(part 1 of 2)
# Autodesk Inventor assembly: 0008-10-02 X Axis
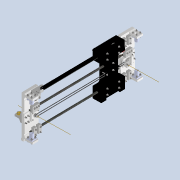
[picture p0: Inventor's stored thumbnail of the model, 180x180]
Saved by Autodesk Inventor 2020 (Build 240168000, 168)
## iProperties
Created: 2021-02-20
Part Number: 0008-10-02 X Axis
Document SubType Name: Assembly
Designer: Iulian Bors
Description: X axis
Author: Iulian Bors
Subject: 10-02
## Documents named in this file (36)
- Z:\I.A.B\Proiecte\0008 I.A.B 3D 2.1 Imprimanta aracet Metal\10 Mecanic\0008-10-02 X Axis.iam
- Z:\I.A.B\Proiecte\0008 I.A.B 3D 2.1 Imprimanta aracet Metal\10 Mecanic\0008-10-006 suport injectomat.ipt
- Z:\I.A.B\Proiecte\0008 I.A.B 3D 2.1 Imprimanta aracet Metal\10 Mecanic\0008-10-1009 LM10uu.ipt
- Z:\I.A.B\Proiecte\0008 I.A.B 3D 2.1 Imprimanta aracet Metal\10 Mecanic\0008-10-007 Contra suport injectomat.ipt
- Z:\I.A.B\Proiecte\0008 I.A.B 3D 2.1 Imprimanta aracet Metal\10 Mecanic\0008-10-008 X Axis suport.ipt
- Z:\I.A.B\Proiecte\0008 I.A.B 3D 2.1 Imprimanta aracet Metal\10 Mecanic\0008-10-1001 NEMA17 - Motor de passo.ipt
- Z:\I.A.B\Proiecte\0008 I.A.B 3D 2.1 Imprimanta aracet Metal\10 Mecanic\0008-10-1011 GT2 Timing Pulley 20 Tooth.ipt
- Z:\I.A.B\Proiecte\0008 I.A.B 3D 2.1 Imprimanta aracet Metal\10 Mecanic\0008-10-009 X Axis suport.ipt
- Z:\I.A.B\Proiecte\0008 I.A.B 3D 2.1 Imprimanta aracet Metal\10 Mecanic\0008-10-010 Fixare AxaX.ipt
- Z:\I.A.B\Proiecte\0008 I.A.B 3D 2.1 Imprimanta aracet Metal\10 Mecanic\0008-10-011 Fixare AxaX Mijloc.ipt
- Z:\I.A.B\Proiecte\0008 I.A.B 3D 2.1 Imprimanta aracet Metal\10 Mecanic\0008-10-012 Intinzator X.ipt
- Z:\I.A.B\Proiecte\0008 I.A.B 3D 2.1 Imprimanta aracet Metal\10 Mecanic\0008-10-1012 16T W6 B3 Without T_Shrinkwrap_1.ipt
- Z:\I.A.B\Proiecte\0008 I.A.B 3D 2.1 Imprimanta aracet Metal\10 Mecanic\0008-10-1013 LMK 10 Bearing.ipt
- Z:\I.A.B\Proiecte\0008 I.A.B 3D 2.1 Imprimanta aracet Metal\10 Mecanic\0008-10-013 Supăort Piulita Axa Z.ipt
- Z:\I.A.B\Proiecte\0008 I.A.B 3D 2.1 Imprimanta aracet Metal\10 Mecanic\0008-10-1004 Piulita.ipt
- Z:\I.A.B\Proiecte\0008 I.A.B 3D 2.1 Imprimanta aracet Metal\10 Mecanic\0008-10-1008 Bara 10_V1.ipt
- Z:\I.A.B\Proiecte\0008 I.A.B 3D 2.1 Imprimanta aracet Metal\20 Electric\0008-20-1003 Switch.ipt
- Z:\I.A.B\Proiecte\0008 I.A.B 3D 2.1 Imprimanta aracet Metal\10 Mecanic\0008-10-046 Fixare axa si port cablu.ipt
- Z:\I.A.B\Proiecte\0008 I.A.B 3D 2.1 Imprimanta aracet Metal\10 Mecanic\0008-10-2000 DIN 6912 - M4 x 25.ipt
- Z:\I.A.B\Proiecte\0008 I.A.B 3D 2.1 Imprimanta aracet Metal\10 Mecanic\0008-10-2002 DIN 125 - A 4.3.ipt
- Z:\I.A.B\Proiecte\0008 I.A.B 3D 2.1 Imprimanta aracet Metal\10 Mecanic\0008-10-2001 DIN 934 - M4 x 0.7.ipt
- Z:\I.A.B\Proiecte\0008 I.A.B 3D 2.1 Imprimanta aracet Metal\10 Mecanic\0008-10-2018 DIN 912 - M4 x 0.7 x 40.ipt
- Z:\I.A.B\Proiecte\0008 I.A.B 3D 2.1 Imprimanta aracet Metal\10 Mecanic\0008-10-2019 DIN 6912 - M4 x 50.ipt
- Z:\I.A.B\Proiecte\0008 I.A.B 3D 2.1 Imprimanta aracet Metal\10 Mecanic\0008-10-2003DIN 6912 - M4 x 35.ipt
- Z:\I.A.B\Proiecte\0008 I.A.B 3D 2.1 Imprimanta aracet Metal\10 Mecanic\0008-10-2006 DIN 7984 - M3 x 16.ipt
- Z:\I.A.B\Proiecte\0008 I.A.B 3D 2.1 Imprimanta aracet Metal\10 Mecanic\0008-10-2009 DIN 555-5 - M3.ipt
- Z:\I.A.B\Proiecte\0008 I.A.B 3D 2.1 Imprimanta aracet Metal\10 Mecanic\0008-10-2020 DIN 7991 - M3  x  16.ipt
- Z:\I.A.B\Proiecte\0008 I.A.B 3D 2.1 Imprimanta aracet Metal\10 Mecanic\0008-10-2005 DIN 125 - A 3.2.ipt
- Z:\I.A.B\Proiecte\0008 I.A.B 3D 2.1 Imprimanta aracet Metal\10 Mecanic\0008-10-2004 DIN 7984 - M3 x 20.ipt
- Z:\I.A.B\Proiecte\0008 I.A.B 3D 2.1 Imprimanta aracet Metal\10 Mecanic\0008-10-2021 DIN 7984 - M5 x 30.ipt
- Z:\I.A.B\Proiecte\0008 I.A.B 3D 2.1 Imprimanta aracet Metal\10 Mecanic\0008-10-2012 DIN 125 - A 5.3.ipt
- Z:\I.A.B\Proiecte\0008 I.A.B 3D 2.1 Imprimanta aracet Metal\10 Mecanic\0008-10-2022 DIN 934 - M5 x 0.8.ipt
- Z:\I.A.B\Proiecte\0008 I.A.B 3D 2.1 Imprimanta aracet Metal\10 Mecanic\0008-10-1023 Compress Spring11.ipt
- Z:\I.A.B\Proiecte\0008 I.A.B 3D 2.1 Imprimanta aracet Metal\10 Mecanic\Synchronous Belts Transmission1.iam
- Z:\I.A.B\Proiecte\0008 I.A.B 3D 2.1 Imprimanta aracet Metal\10 Mecanic\0008-10-1025 Wire chain.ipt
- Z:\I.A.B\Proiecte\0008 I.A.B 3D 2.1 Imprimanta aracet Metal\10 Mecanic\0008-10-04 Z axis_Shrinkwrap.ipt
## Components (326 placed, 35 different names)
1. 0008-10-006 suport injectomat.ipt:1 — Flush:3, Flush:4, Mate:8, Mate:9, Flush:5, Flush:6, Angle:2, Mate:17, Mate:23, Insert:178, Insert:197, Insert:198, Insert:199, Insert:200, Insert:201, Insert:202, Insert:212, Insert:213, Insert:214
2. 0008-10-1009 LM10uu.ipt:2 — Flush:1, Mate:5, Mate:8
3. 0008-10-1009 LM10uu.ipt:3 — Mate:5, Flush:121
4. 0008-10-1009 LM10uu.ipt:4 — Flush:4, Mate:6, Mate:9
5. 0008-10-1009 LM10uu.ipt:5 — Flush:3, Mate:6
6. 0008-10-007 Contra suport injectomat.ipt:6 — Flush:5, Flush:6, Mate:23, Flush:121, Flush:122, Insert:234, Insert:238, Mate:199, Flush:130, Insert:312, Insert:313, Flush:1
7. 0008-10-1008 Bara 10_V1.ipt:7
8. 0008-10-1008 Bara 10_V1.ipt:8 — Mate:188, Mate:189, Mate:191, Mate:192
9. 0008-10-009 X Axis suport.ipt:9 — Angle:2, Flush:10, Mate:21, Mate:22, Angle:3, Flush:26, Flush:27, Angle:4, Angle:5, Mate:26, Mate:27, Flush:32, Flush:34, Mate:38, Flush:36, Flush:37, Mate:164, Angle:28, Flush:127, Mate:194, Insert:49, Insert:50, Insert:51, Insert:52, Insert:140, Insert:141, Insert:142, Insert:143, Insert:156, Insert:157, Insert:158, Insert:159, Insert:172, Insert:173, Insert:174, Insert:289, Insert:290, Insert:291, Insert:292
10. 0008-10-008 X Axis suport.ipt:10 — Flush:10, Mate:21, Mate:30, Mate:31, Mate:33, Mate:34, Mate:35, Insert:21, Mate:172, Angle:25, Angle:29, Flush:128, Angle:30, Insert:65, Insert:66, Insert:67, Insert:68, Mate:196, Insert:91, Insert:98, Insert:99, Insert:109, Insert:110, Insert:111, Insert:124, Insert:125, Insert:126, Insert:127, Insert:302, Insert:303, Mate:197
11. 0008-10-1001 NEMA17 - Motor de passo.ipt:11 — Insert:1, Mate:22, Mate:26, Mate:27
12. 0008-10-1009 LM10uu.ipt:12 — Mate:17, Flush:122
13. 0008-10-1008 Bara 10_V1.ipt:13
14. 0008-10-1011 GT2 Timing Pulley 20 Tooth.ipt:14 — Insert:1, Flush:29, Flush:30, Angle:5
15. 0008-10-012 Intinzator X.ipt:15 — Flush:29, Insert:2, Angle:30, Insert:293, Insert:294
16. 0008-10-1012 16T W6 B3 Without T_Shrinkwrap_1.ipt:16 — Insert:2, Flush:30
17. 0008-10-1013 LMK 10 Bearing.ipt:17 — Mate:29, Angle:6, Mate:164
18. 0008-10-1013 LMK 10 Bearing.ipt:18 — Mate:33, Mate:34, Mate:35, Mate:202
19. 0008-10-1013 LMK 10 Bearing.ipt:19 — Mate:30, Mate:31, Angle:25, Insert:81, Insert:82, Insert:83, Insert:84
20. 0008-10-1013 LMK 10 Bearing.ipt:20 — Flush:32, Mate:29, Flush:34, Angle:6, Mate:194, Insert:23, Mate:195, Insert:35, Insert:36
21. 0008-10-046 Fixare axa si port cablu.ipt:21 — Angle:3, Flush:26, Insert:283, Insert:284, Insert:308, Insert:309, Mate:200, Flush:131, Flush:132
22. 0008-10-013 Supăort Piulita Axa Z.ipt:22 — Mate:38, Flush:36, Mate:39, Mate:40, Flush:37, Flush:38, Insert:218, Insert:228, Insert:229, Insert:230
23. 0008-10-1004 Piulita.ipt:23 — Mate:39, Mate:40, Flush:38, Insert:256, Insert:260, Insert:261, Insert:262
24. 0008-10-013 Supăort Piulita Axa Z.ipt:24 — Insert:21, Mate:172, Mate:173, Mate:174, Insert:251, Insert:252, Insert:253, Insert:254
25. 0008-10-1004 Piulita.ipt:25 — Mate:173, Mate:174, Insert:267, Insert:268, Insert:269, Insert:270, Mate:201
26. 0008-20-1003 Switch.ipt:28 — Mate:199, Flush:130, Insert:310, Insert:311
27. 0008-10-010 Fixare AxaX.ipt:29 — Mate:188, Angle:28, Flush:127, Mate:190
28. 0008-10-010 Fixare AxaX.ipt:30 — Mate:189, Mate:190
29. 0008-10-2020 DIN 7991 - M3  x  16.ipt:318 — Insert:309
30. 0008-10-2009 DIN 555-5 - M3.ipt:319
31. 0008-10-2005 DIN 125 - A 3.2.ipt:320
32. 0008-10-2020 DIN 7991 - M3  x  16.ipt:321 — Insert:308
33. 0008-10-2009 DIN 555-5 - M3.ipt:322
34. 0008-10-2005 DIN 125 - A 3.2.ipt:323
35. Synchronous Belts Transmission1.iam:324 [sub-assembly]
36. 0008-10-1025 Wire chain.ipt:325 — Mate:200, Flush:131, Flush:132
37. 0008-10-04 Z axis_Shrinkwrap.ipt:326 — Mate:201, Mate:202
38. 0008-10-2022 DIN 934 - M5 x 0.8.ipt:35 — Insert:295
39. 0008-10-2018 DIN 912 - M4 x 0.7 x 40.ipt:36 — Mate:198
40. 0008-10-2002 DIN 125 - A 4.3.ipt:37
41. 0008-10-2001 DIN 934 - M4 x 0.7.ipt:38
42. 0008-10-2002 DIN 125 - A 4.3.ipt:39 — Insert:302
43. 0008-10-2018 DIN 912 - M4 x 0.7 x 40.ipt:40
44. 0008-10-2002 DIN 125 - A 4.3.ipt:41
45. 0008-10-2001 DIN 934 - M4 x 0.7.ipt:42
46. 0008-10-2002 DIN 125 - A 4.3.ipt:43 — Insert:303
47. 0008-10-2003DIN 6912 - M4 x 35.ipt:44
48. 0008-10-2002 DIN 125 - A 4.3.ipt:45 — Insert:230
49. 0008-10-2002 DIN 125 - A 4.3.ipt:46
50. 0008-10-2001 DIN 934 - M4 x 0.7.ipt:47
51. 0008-10-2003DIN 6912 - M4 x 35.ipt:48
52. 0008-10-2002 DIN 125 - A 4.3.ipt:49 — Insert:229
53. 0008-10-2002 DIN 125 - A 4.3.ipt:50
54. 0008-10-2001 DIN 934 - M4 x 0.7.ipt:51
55. 0008-10-2003DIN 6912 - M4 x 35.ipt:52
56. 0008-10-2002 DIN 125 - A 4.3.ipt:53 — Insert:228
57. 0008-10-2002 DIN 125 - A 4.3.ipt:54
58. 0008-10-2001 DIN 934 - M4 x 0.7.ipt:55
59. 0008-10-2003DIN 6912 - M4 x 35.ipt:56
60. 0008-10-2002 DIN 125 - A 4.3.ipt:57 — Insert:234
61. 0008-10-2002 DIN 125 - A 4.3.ipt:58
62. 0008-10-2001 DIN 934 - M4 x 0.7.ipt:59
63. 0008-10-2003DIN 6912 - M4 x 35.ipt:60
64. 0008-10-2002 DIN 125 - A 4.3.ipt:61 — Insert:238
65. 0008-10-2002 DIN 125 - A 4.3.ipt:62
66. 0008-10-2001 DIN 934 - M4 x 0.7.ipt:63
67. 0008-10-2003DIN 6912 - M4 x 35.ipt:64
68. 0008-10-2002 DIN 125 - A 4.3.ipt:65 — Insert:253
69. 0008-10-2002 DIN 125 - A 4.3.ipt:66
70. 0008-10-2001 DIN 934 - M4 x 0.7.ipt:67
71. 0008-10-2003DIN 6912 - M4 x 35.ipt:68
72. 0008-10-2002 DIN 125 - A 4.3.ipt:69 — Insert:254
73. 0008-10-2002 DIN 125 - A 4.3.ipt:70
74. 0008-10-2001 DIN 934 - M4 x 0.7.ipt:71
75. 0008-10-2003DIN 6912 - M4 x 35.ipt:72
76. 0008-10-2002 DIN 125 - A 4.3.ipt:73 — Insert:252
77. 0008-10-2002 DIN 125 - A 4.3.ipt:74
78. 0008-10-2001 DIN 934 - M4 x 0.7.ipt:75
79. 0008-10-2003DIN 6912 - M4 x 35.ipt:76
80. 0008-10-2002 DIN 125 - A 4.3.ipt:77 — Insert:251
81. 0008-10-2002 DIN 125 - A 4.3.ipt:78
82. 0008-10-2001 DIN 934 - M4 x 0.7.ipt:79
83. 0008-10-2006 DIN 7984 - M3 x 16.ipt:80 — Insert:256
84. 0008-10-2009 DIN 555-5 - M3.ipt:81
85. 0008-10-2006 DIN 7984 - M3 x 16.ipt:82 — Insert:261
86. 0008-10-2009 DIN 555-5 - M3.ipt:83
87. 0008-10-2006 DIN 7984 - M3 x 16.ipt:84 — Insert:260
88. 0008-10-2009 DIN 555-5 - M3.ipt:85
89. 0008-10-2006 DIN 7984 - M3 x 16.ipt:86 — Insert:262
90. 0008-10-2009 DIN 555-5 - M3.ipt:87
91. 0008-10-2006 DIN 7984 - M3 x 16.ipt:88 — Insert:268
92. 0008-10-2009 DIN 555-5 - M3.ipt:89
93. 0008-10-2006 DIN 7984 - M3 x 16.ipt:90 — Insert:269
94. 0008-10-2009 DIN 555-5 - M3.ipt:91
95. 0008-10-2006 DIN 7984 - M3 x 16.ipt:92 — Insert:270
96. 0008-10-2009 DIN 555-5 - M3.ipt:93
97. 0008-10-2006 DIN 7984 - M3 x 16.ipt:94 — Insert:267
98. 0008-10-2009 DIN 555-5 - M3.ipt:95
99. 0008-10-2006 DIN 7984 - M3 x 16.ipt:96 — Insert:310
100. 0008-10-2006 DIN 7984 - M3 x 16.ipt:97 — Insert:311
101. 0008-10-2020 DIN 7991 - M3  x  16.ipt:98 — Insert:274, Insert:312
102. 0008-10-2009 DIN 555-5 - M3.ipt:99 — Insert:274
103. 0008-10-2005 DIN 125 - A 3.2.ipt:100
104. 0008-10-2020 DIN 7991 - M3  x  16.ipt:101 — Insert:313
105. 0008-10-2009 DIN 555-5 - M3.ipt:102
106. 0008-10-2005 DIN 125 - A 3.2.ipt:103
107. 0008-10-2020 DIN 7991 - M3  x  16.ipt:104 — Insert:283
108. 0008-10-2009 DIN 555-5 - M3.ipt:105
109. 0008-10-2005 DIN 125 - A 3.2.ipt:106
110. 0008-10-2020 DIN 7991 - M3  x  16.ipt:107 — Insert:284
111. 0008-10-2009 DIN 555-5 - M3.ipt:108
112. 0008-10-2005 DIN 125 - A 3.2.ipt:109
113. 0008-10-2004 DIN 7984 - M3 x 20.ipt:110 — Insert:285
114. 0008-10-2005 DIN 125 - A 3.2.ipt:111 — Insert:285, Insert:292
115. 0008-10-2004 DIN 7984 - M3 x 20.ipt:112
116. 0008-10-2005 DIN 125 - A 3.2.ipt:113 — Insert:291
117. 0008-10-2004 DIN 7984 - M3 x 20.ipt:114
118. 0008-10-2005 DIN 125 - A 3.2.ipt:115 — Insert:290
119. 0008-10-2004 DIN 7984 - M3 x 20.ipt:116
120. 0008-10-2005 DIN 125 - A 3.2.ipt:117 — Insert:289
121. 0008-10-2021 DIN 7984 - M5 x 30.ipt:118 — Insert:293
122. 0008-10-2012 DIN 125 - A 5.3.ipt:119 — Insert:294, Insert:295
123. 0008-10-2000 DIN 6912 - M4 x 25.ipt:120 — Insert:22, Insert:25
124. 0008-10-2002 DIN 125 - A 4.3.ipt:121 — Insert:22, Insert:23
125. 0008-10-2002 DIN 125 - A 4.3.ipt:122 — Insert:24
126. 0008-10-2001 DIN 934 - M4 x 0.7.ipt:123 — Insert:24, Insert:25
127. 0008-10-2000 DIN 6912 - M4 x 25.ipt:124
128. 0008-10-2002 DIN 125 - A 4.3.ipt:125 — Mate:195
129. 0008-10-2002 DIN 125 - A 4.3.ipt:126
130. 0008-10-2001 DIN 934 - M4 x 0.7.ipt:127
131. 0008-10-2000 DIN 6912 - M4 x 25.ipt:128
132. 0008-10-2002 DIN 125 - A 4.3.ipt:129 — Insert:36
133. 0008-10-2002 DIN 125 - A 4.3.ipt:130
134. 0008-10-2001 DIN 934 - M4 x 0.7.ipt:131
135. 0008-10-2000 DIN 6912 - M4 x 25.ipt:132
136. 0008-10-2002 DIN 125 - A 4.3.ipt:133 — Insert:35
137. 0008-10-2002 DIN 125 - A 4.3.ipt:134
138. 0008-10-2001 DIN 934 - M4 x 0.7.ipt:135
139. 0008-10-2000 DIN 6912 - M4 x 25.ipt:136
140. 0008-10-2002 DIN 125 - A 4.3.ipt:137 — Insert:50
141. 0008-10-2002 DIN 125 - A 4.3.ipt:138
142. 0008-10-2001 DIN 934 - M4 x 0.7.ipt:139
143. 0008-10-2000 DIN 6912 - M4 x 25.ipt:140
144. 0008-10-2002 DIN 125 - A 4.3.ipt:141 — Insert:52
145. 0008-10-2002 DIN 125 - A 4.3.ipt:142
146. 0008-10-2001 DIN 934 - M4 x 0.7.ipt:143
147. 0008-10-2000 DIN 6912 - M4 x 25.ipt:144
148. 0008-10-2002 DIN 125 - A 4.3.ipt:145 — Insert:51
149. 0008-10-2002 DIN 125 - A 4.3.ipt:146
150. 0008-10-2001 DIN 934 - M4 x 0.7.ipt:147
151. 0008-10-2000 DIN 6912 - M4 x 25.ipt:148
152. 0008-10-2002 DIN 125 - A 4.3.ipt:149 — Insert:49
153. 0008-10-2002 DIN 125 - A 4.3.ipt:150
154. 0008-10-2001 DIN 934 - M4 x 0.7.ipt:151
155. 0008-10-2000 DIN 6912 - M4 x 25.ipt:152
156. 0008-10-2002 DIN 125 - A 4.3.ipt:153 — Insert:66
157. 0008-10-2002 DIN 125 - A 4.3.ipt:154
158. 0008-10-2001 DIN 934 - M4 x 0.7.ipt:155
159. 0008-10-2000 DIN 6912 - M4 x 25.ipt:156
160. 0008-10-2002 DIN 125 - A 4.3.ipt:157 — Insert:65
161. 0008-10-2002 DIN 125 - A 4.3.ipt:158
162. 0008-10-2001 DIN 934 - M4 x 0.7.ipt:159
163. 0008-10-2000 DIN 6912 - M4 x 25.ipt:160
164. 0008-10-2002 DIN 125 - A 4.3.ipt:161 — Insert:67
165. 0008-10-2002 DIN 125 - A 4.3.ipt:162
166. 0008-10-2001 DIN 934 - M4 x 0.7.ipt:163
167. 0008-10-2000 DIN 6912 - M4 x 25.ipt:164
168. 0008-10-2002 DIN 125 - A 4.3.ipt:165 — Insert:68
169. 0008-10-2002 DIN 125 - A 4.3.ipt:166
170. 0008-10-2001 DIN 934 - M4 x 0.7.ipt:167
171. 0008-10-2000 DIN 6912 - M4 x 25.ipt:168
172. 0008-10-2002 DIN 125 - A 4.3.ipt:169 — Insert:84
173. 0008-10-2002 DIN 125 - A 4.3.ipt:170
174. 0008-10-2001 DIN 934 - M4 x 0.7.ipt:171
175. 0008-10-2000 DIN 6912 - M4 x 25.ipt:172
176. 0008-10-2002 DIN 125 - A 4.3.ipt:173 — Insert:83
177. 0008-10-2002 DIN 125 - A 4.3.ipt:174
178. 0008-10-2001 DIN 934 - M4 x 0.7.ipt:175
179. 0008-10-2000 DIN 6912 - M4 x 25.ipt:176
180. 0008-10-2002 DIN 125 - A 4.3.ipt:177 — Insert:82
181. 0008-10-2002 DIN 125 - A 4.3.ipt:178
182. 0008-10-2001 DIN 934 - M4 x 0.7.ipt:179
183. 0008-10-2000 DIN 6912 - M4 x 25.ipt:180
184. 0008-10-2002 DIN 125 - A 4.3.ipt:181 — Insert:81
185. 0008-10-2002 DIN 125 - A 4.3.ipt:182
186. 0008-10-2001 DIN 934 - M4 x 0.7.ipt:183
187. 0008-10-2018 DIN 912 - M4 x 0.7 x 40.ipt:184 — Insert:86, Insert:87
188. 0008-10-2002 DIN 125 - A 4.3.ipt:185
189. 0008-10-2001 DIN 934 - M4 x 0.7.ipt:186 — Insert:87
190. 0008-10-2002 DIN 125 - A 4.3.ipt:187 — Insert:86, Mate:196
191. 0008-10-2018 DIN 912 - M4 x 0.7 x 40.ipt:188
192. 0008-10-2002 DIN 125 - A 4.3.ipt:189
193. 0008-10-2001 DIN 934 - M4 x 0.7.ipt:190
194. 0008-10-2002 DIN 125 - A 4.3.ipt:191 — Insert:91
195. 0008-10-2018 DIN 912 - M4 x 0.7 x 40.ipt:192
196. 0008-10-2002 DIN 125 - A 4.3.ipt:193
197. 0008-10-2001 DIN 934 - M4 x 0.7.ipt:194
198. 0008-10-2002 DIN 125 - A 4.3.ipt:195 — Insert:98
199. 0008-10-2018 DIN 912 - M4 x 0.7 x 40.ipt:196
200. 0008-10-2002 DIN 125 - A 4.3.ipt:197
201. 0008-10-2001 DIN 934 - M4 x 0.7.ipt:198
202. 0008-10-2002 DIN 125 - A 4.3.ipt:199 — Insert:99
203. 0008-10-2018 DIN 912 - M4 x 0.7 x 40.ipt:200
204. 0008-10-2002 DIN 125 - A 4.3.ipt:201
205. 0008-10-2001 DIN 934 - M4 x 0.7.ipt:202
206. 0008-10-2002 DIN 125 - A 4.3.ipt:203 — Insert:110
207. 0008-10-2018 DIN 912 - M4 x 0.7 x 40.ipt:204
208. 0008-10-2002 DIN 125 - A 4.3.ipt:205
209. 0008-10-2001 DIN 934 - M4 x 0.7.ipt:206
210. 0008-10-2002 DIN 125 - A 4.3.ipt:207 — Insert:111
211. 0008-10-2018 DIN 912 - M4 x 0.7 x 40.ipt:208
212. 0008-10-2002 DIN 125 - A 4.3.ipt:209
213. 0008-10-2001 DIN 934 - M4 x 0.7.ipt:210
214. 0008-10-2002 DIN 125 - A 4.3.ipt:211 — Insert:109
215. 0008-10-2018 DIN 912 - M4 x 0.7 x 40.ipt:212
216. 0008-10-2002 DIN 125 - A 4.3.ipt:213
217. 0008-10-2001 DIN 934 - M4 x 0.7.ipt:214
218. 0008-10-2002 DIN 125 - A 4.3.ipt:215 — Insert:126
219. 0008-10-2018 DIN 912 - M4 x 0.7 x 40.ipt:216
220. 0008-10-2002 DIN 125 - A 4.3.ipt:217
221. 0008-10-2001 DIN 934 - M4 x 0.7.ipt:218
222. 0008-10-2002 DIN 125 - A 4.3.ipt:219 — Insert:124
223. 0008-10-2018 DIN 912 - M4 x 0.7 x 40.ipt:220
224. 0008-10-2002 DIN 125 - A 4.3.ipt:221
225. 0008-10-2001 DIN 934 - M4 x 0.7.ipt:222
226. 0008-10-2002 DIN 125 - A 4.3.ipt:223 — Insert:125
227. 0008-10-2018 DIN 912 - M4 x 0.7 x 40.ipt:224
228. 0008-10-2002 DIN 125 - A 4.3.ipt:225
229. 0008-10-2001 DIN 934 - M4 x 0.7.ipt:226
230. 0008-10-2002 DIN 125 - A 4.3.ipt:227 — Insert:127
231. 0008-10-2018 DIN 912 - M4 x 0.7 x 40.ipt:228
232. 0008-10-2002 DIN 125 - A 4.3.ipt:229
233. 0008-10-2001 DIN 934 - M4 x 0.7.ipt:230
234. 0008-10-2002 DIN 125 - A 4.3.ipt:231 — Insert:141
235. 0008-10-2018 DIN 912 - M4 x 0.7 x 40.ipt:232
236. 0008-10-2002 DIN 125 - A 4.3.ipt:233
237. 0008-10-2001 DIN 934 - M4 x 0.7.ipt:234
238. 0008-10-2002 DIN 125 - A 4.3.ipt:235 — Insert:142
239. 0008-10-2018 DIN 912 - M4 x 0.7 x 40.ipt:236
240. 0008-10-2002 DIN 125 - A 4.3.ipt:237
241. 0008-10-2001 DIN 934 - M4 x 0.7.ipt:238
242. 0008-10-2002 DIN 125 - A 4.3.ipt:239 — Insert:143
243. 0008-10-2018 DIN 912 - M4 x 0.7 x 40.ipt:240
244. 0008-10-2002 DIN 125 - A 4.3.ipt:241
245. 0008-10-2001 DIN 934 - M4 x 0.7.ipt:242
246. 0008-10-2002 DIN 125 - A 4.3.ipt:243 — Insert:140
247. 0008-10-2018 DIN 912 - M4 x 0.7 x 40.ipt:244
248. 0008-10-2002 DIN 125 - A 4.3.ipt:245
249. 0008-10-2001 DIN 934 - M4 x 0.7.ipt:246
250. 0008-10-2002 DIN 125 - A 4.3.ipt:247 — Insert:156
251. 0008-10-2018 DIN 912 - M4 x 0.7 x 40.ipt:248
252. 0008-10-2002 DIN 125 - A 4.3.ipt:249
253. 0008-10-2001 DIN 934 - M4 x 0.7.ipt:250
254. 0008-10-2002 DIN 125 - A 4.3.ipt:251 — Insert:157
255. 0008-10-2018 DIN 912 - M4 x 0.7 x 40.ipt:252
256. 0008-10-2002 DIN 125 - A 4.3.ipt:253
257. 0008-10-2001 DIN 934 - M4 x 0.7.ipt:254
258. 0008-10-2002 DIN 125 - A 4.3.ipt:255 — Insert:158
259. 0008-10-2018 DIN 912 - M4 x 0.7 x 40.ipt:256
260. 0008-10-2002 DIN 125 - A 4.3.ipt:257
261. 0008-10-2001 DIN 934 - M4 x 0.7.ipt:258
262. 0008-10-2002 DIN 125 - A 4.3.ipt:259 — Insert:159
263. 0008-10-2018 DIN 912 - M4 x 0.7 x 40.ipt:260
264. 0008-10-2002 DIN 125 - A 4.3.ipt:261
265. 0008-10-2001 DIN 934 - M4 x 0.7.ipt:262
266. 0008-10-2002 DIN 125 - A 4.3.ipt:263 — Insert:173
267. 0008-10-2018 DIN 912 - M4 x 0.7 x 40.ipt:264
268. 0008-10-2002 DIN 125 - A 4.3.ipt:265
269. 0008-10-2001 DIN 934 - M4 x 0.7.ipt:266
270. 0008-10-2002 DIN 125 - A 4.3.ipt:267 — Insert:174
271. 0008-10-2018 DIN 912 - M4 x 0.7 x 40.ipt:268
272. 0008-10-2002 DIN 125 - A 4.3.ipt:269
273. 0008-10-2001 DIN 934 - M4 x 0.7.ipt:270
274. 0008-10-2002 DIN 125 - A 4.3.ipt:271 — Insert:172
275. 0008-10-2019 DIN 6912 - M4 x 50.ipt:272 — Insert:175, Insert:177
276. 0008-10-2002 DIN 125 - A 4.3.ipt:273 — Insert:175, Insert:178
277. 0008-10-2002 DIN 125 - A 4.3.ipt:274 — Insert:176
278. 0008-10-2001 DIN 934 - M4 x 0.7.ipt:275 — Insert:176, Insert:177
279. 0008-10-2019 DIN 6912 - M4 x 50.ipt:276
280. 0008-10-2002 DIN 125 - A 4.3.ipt:277 — Insert:197
281. 0008-10-2002 DIN 125 - A 4.3.ipt:278
282. 0008-10-2001 DIN 934 - M4 x 0.7.ipt:279
283. 0008-10-2019 DIN 6912 - M4 x 50.ipt:280
284. 0008-10-2002 DIN 125 - A 4.3.ipt:281 — Insert:199
285. 0008-10-2002 DIN 125 - A 4.3.ipt:282
286. 0008-10-2001 DIN 934 - M4 x 0.7.ipt:283
287. 0008-10-2019 DIN 6912 - M4 x 50.ipt:284
288. 0008-10-2002 DIN 125 - A 4.3.ipt:285 — Insert:198
289. 0008-10-2002 DIN 125 - A 4.3.ipt:286
290. 0008-10-2001 DIN 934 - M4 x 0.7.ipt:287
291. 0008-10-2019 DIN 6912 - M4 x 50.ipt:288
292. 0008-10-2002 DIN 125 - A 4.3.ipt:289 — Insert:200
293. 0008-10-2002 DIN 125 - A 4.3.ipt:290
294. 0008-10-2001 DIN 934 - M4 x 0.7.ipt:291
295. 0008-10-2019 DIN 6912 - M4 x 50.ipt:292
296. 0008-10-2002 DIN 125 - A 4.3.ipt:293 — Insert:201
297. 0008-10-2002 DIN 125 - A 4.3.ipt:294
298. 0008-10-2001 DIN 934 - M4 x 0.7.ipt:295
299. 0008-10-2019 DIN 6912 - M4 x 50.ipt:296
300. 0008-10-2002 DIN 125 - A 4.3.ipt:297 — Insert:202
301. 0008-10-2002 DIN 125 - A 4.3.ipt:298
302. 0008-10-2001 DIN 934 - M4 x 0.7.ipt:299
303. 0008-10-2019 DIN 6912 - M4 x 50.ipt:300
304. 0008-10-2002 DIN 125 - A 4.3.ipt:301 — Insert:213
305. 0008-10-2002 DIN 125 - A 4.3.ipt:302
306. 0008-10-2001 DIN 934 - M4 x 0.7.ipt:303
307. 0008-10-2019 DIN 6912 - M4 x 50.ipt:304
308. 0008-10-2002 DIN 125 - A 4.3.ipt:305 — Insert:212
309. 0008-10-2002 DIN 125 - A 4.3.ipt:306
310. 0008-10-2001 DIN 934 - M4 x 0.7.ipt:307
311. 0008-10-2019 DIN 6912 - M4 x 50.ipt:308
312. 0008-10-2002 DIN 125 - A 4.3.ipt:309 — Insert:214
313. 0008-10-2002 DIN 125 - A 4.3.ipt:310
314. 0008-10-2001 DIN 934 - M4 x 0.7.ipt:311
315. 0008-10-2003DIN 6912 - M4 x 35.ipt:312 — Insert:215, Insert:217
316. 0008-10-2002 DIN 125 - A 4.3.ipt:313 — Insert:215, Insert:218
317. 0008-10-2002 DIN 125 - A 4.3.ipt:314 — Insert:216
318. 0008-10-2001 DIN 934 - M4 x 0.7.ipt:315 — Insert:216, Insert:217
319. 0008-10-011 Fixare AxaX Mijloc.ipt:26 — Flush:27, Angle:4
320. 0008-10-011 Fixare AxaX Mijloc.ipt:27
321. 0008-10-010 Fixare AxaX.ipt:31 — Mate:191, Angle:29, Flush:128, Flush:129, Mate:193
322. 0008-10-010 Fixare AxaX.ipt:32 — Mate:192, Flush:129, Mate:193
323. 0008-10-010 Fixare AxaX.ipt:33
324. 0008-10-010 Fixare AxaX.ipt:34
325. 0008-10-1023 Compress Spring11.ipt:316 — Mate:197, Mate:198
326. 0008-10-1023 Compress Spring11.ipt:317
## Component patterns: (2 elements, first: 0008-10-011 Fixare AxaX Mijloc.ipt:26), (2 elements, first: 0008-10-010 Fixare AxaX.ipt:31 + 0008-10-010 Fixare AxaX.ipt:32), (2 elements, first: 0008-10-1023 Compress Spring11.ipt:316)
## Relationships (368: Insert 288, Mate 43, Flush 27, Angle 9, Tangent 1)
- Flush:1 (20 mm): 0008-10-1009 LM10uu.ipt:2 ↔ 0008-10-007 Contra suport injectomat.ipt:6
- Mate:5: 0008-10-1009 LM10uu.ipt:2 ↔ 0008-10-1009 LM10uu.ipt:3
- Flush:3 (20 mm): 0008-10-006 suport injectomat.ipt:1 ↔ 0008-10-1009 LM10uu.ipt:5
- Flush:4 (20 mm): 0008-10-006 suport injectomat.ipt:1 ↔ 0008-10-1009 LM10uu.ipt:4
- Mate:6: 0008-10-1009 LM10uu.ipt:4 ↔ 0008-10-1009 LM10uu.ipt:5
- Mate:8: 0008-10-006 suport injectomat.ipt:1 ↔ 0008-10-1009 LM10uu.ipt:2
- Mate:9: 0008-10-006 suport injectomat.ipt:1 ↔ 0008-10-1009 LM10uu.ipt:4
- Flush:5: 0008-10-006 suport injectomat.ipt:1 ↔ 0008-10-007 Contra suport injectomat.ipt:6
- Flush:6: 0008-10-006 suport injectomat.ipt:1 ↔ 0008-10-007 Contra suport injectomat.ipt:6
- [Mate]: 0008-10-1009 LM10uu.ipt:3 ↔ 0008-10-1008 Bara 10_V1.ipt:7
- [Mate]: 0008-10-1009 LM10uu.ipt:5 ↔ 0008-10-1008 Bara 10_V1.ipt:8
- [Flush]: 0008-10-1008 Bara 10_V1.ipt:7 ↔ 0008-10-1008 Bara 10_V1.ipt:8
- [Tangent] (-3 mm): 0008-10-1008 Bara 10_V1.ipt:7 ↔ 0008-10-009 X Axis suport.ipt:9
- Angle:2 (0 deg): 0008-10-006 suport injectomat.ipt:1 ↔ 0008-10-009 X Axis suport.ipt:9
- [Flush] (-30 mm): 0008-10-1008 Bara 10_V1.ipt:7 ↔ 0008-10-009 X Axis suport.ipt:9
- Flush:10: 0008-10-009 X Axis suport.ipt:9 ↔ 0008-10-008 X Axis suport.ipt:10
- [Flush] (-30 mm): 0008-10-1008 Bara 10_V1.ipt:7 ↔ 0008-10-008 X Axis suport.ipt:10
- Mate:21: 0008-10-009 X Axis suport.ipt:9 ↔ 0008-10-008 X Axis suport.ipt:10
- Mate:17: 0008-10-006 suport injectomat.ipt:1 ↔ 0008-10-1009 LM10uu.ipt:12
- Insert:1: 0008-10-1001 NEMA17 - Motor de passo.ipt:11 ↔ 0008-10-1011 GT2 Timing Pulley 20 Tooth.ipt:14
- Mate:22 (-10 mm): 0008-10-009 X Axis suport.ipt:9 ↔ 0008-10-1001 NEMA17 - Motor de passo.ipt:11
- Mate:23 (2 mm): 0008-10-006 suport injectomat.ipt:1 ↔ 0008-10-007 Contra suport injectomat.ipt:6
- [Flush]: 0008-10-1008 Bara 10_V1.ipt:7 ↔ 0008-10-1008 Bara 10_V1.ipt:13
- [Mate]: 0008-10-1008 Bara 10_V1.ipt:7 ↔ 0008-10-046 Fixare axa si port cablu.ipt:21
- Angle:3 (0 deg): 0008-10-009 X Axis suport.ipt:9 ↔ 0008-10-046 Fixare axa si port cablu.ipt:21
- Flush:26 (35 mm): 0008-10-009 X Axis suport.ipt:9 ↔ 0008-10-046 Fixare axa si port cablu.ipt:21
- [Mate]: 0008-10-1008 Bara 10_V1.ipt:13 ↔ 0008-10-011 Fixare AxaX Mijloc.ipt:26
- Flush:27 (30 mm): 0008-10-009 X Axis suport.ipt:9 ↔ 0008-10-011 Fixare AxaX Mijloc.ipt:26
- Angle:4 (0 deg): 0008-10-009 X Axis suport.ipt:9 ↔ 0008-10-011 Fixare AxaX Mijloc.ipt:26
- Flush:29: 0008-10-1011 GT2 Timing Pulley 20 Tooth.ipt:14 ↔ 0008-10-012 Intinzator X.ipt:15
- Insert:2 (0.25 mm): 0008-10-012 Intinzator X.ipt:15 ↔ 0008-10-1012 16T W6 B3 Without T_Shrinkwrap_1.ipt:16
- Flush:30: 0008-10-1011 GT2 Timing Pulley 20 Tooth.ipt:14 ↔ 0008-10-1012 16T W6 B3 Without T_Shrinkwrap_1.ipt:16
- Angle:5 (0 deg): 0008-10-009 X Axis suport.ipt:9 ↔ 0008-10-1011 GT2 Timing Pulley 20 Tooth.ipt:14
- Mate:26 (1 mm): 0008-10-009 X Axis suport.ipt:9 ↔ 0008-10-1001 NEMA17 - Motor de passo.ipt:11
- Mate:27 (1 mm): 0008-10-009 X Axis suport.ipt:9 ↔ 0008-10-1001 NEMA17 - Motor de passo.ipt:11
- Flush:32 (15 mm): 0008-10-009 X Axis suport.ipt:9 ↔ 0008-10-1013 LMK 10 Bearing.ipt:20
- Mate:29: 0008-10-1013 LMK 10 Bearing.ipt:17 ↔ 0008-10-1013 LMK 10 Bearing.ipt:20
- Flush:34: 0008-10-009 X Axis suport.ipt:9 ↔ 0008-10-1013 LMK 10 Bearing.ipt:20
- Angle:6 (0 deg): 0008-10-1013 LMK 10 Bearing.ipt:17 ↔ 0008-10-1013 LMK 10 Bearing.ipt:20
- Mate:30: 0008-10-008 X Axis suport.ipt:10 ↔ 0008-10-1013 LMK 10 Bearing.ipt:19
- Mate:31: 0008-10-008 X Axis suport.ipt:10 ↔ 0008-10-1013 LMK 10 Bearing.ipt:19
- Mate:33: 0008-10-008 X Axis suport.ipt:10 ↔ 0008-10-1013 LMK 10 Bearing.ipt:18
- Mate:34: 0008-10-008 X Axis suport.ipt:10 ↔ 0008-10-1013 LMK 10 Bearing.ipt:18
- Mate:35: 0008-10-008 X Axis suport.ipt:10 ↔ 0008-10-1013 LMK 10 Bearing.ipt:18
- Mate:38: 0008-10-009 X Axis suport.ipt:9 ↔ 0008-10-013 Supăort Piulita Axa Z.ipt:22
- Flush:36: 0008-10-009 X Axis suport.ipt:9 ↔ 0008-10-013 Supăort Piulita Axa Z.ipt:22
- Mate:39: 0008-10-013 Supăort Piulita Axa Z.ipt:22 ↔ 0008-10-1004 Piulita.ipt:23
- Mate:40 (-12 mm): 0008-10-013 Supăort Piulita Axa Z.ipt:22 ↔ 0008-10-1004 Piulita.ipt:23
- Flush:37 (80 mm): 0008-10-009 X Axis suport.ipt:9 ↔ 0008-10-013 Supăort Piulita Axa Z.ipt:22
- Flush:38 (15 mm): 0008-10-013 Supăort Piulita Axa Z.ipt:22 ↔ 0008-10-1004 Piulita.ipt:23
- [Mate]: 0008-10-1008 Bara 10_V1.ipt:7 ↔ 0008-10-009 X Axis suport.ipt:9
- Mate:164: 0008-10-009 X Axis suport.ipt:9 ↔ 0008-10-1013 LMK 10 Bearing.ipt:17
- Insert:21: 0008-10-008 X Axis suport.ipt:10 ↔ 0008-10-013 Supăort Piulita Axa Z.ipt:24
- Mate:172: 0008-10-008 X Axis suport.ipt:10 ↔ 0008-10-013 Supăort Piulita Axa Z.ipt:24
- Mate:173: 0008-10-013 Supăort Piulita Axa Z.ipt:24 ↔ 0008-10-1004 Piulita.ipt:25
- Mate:174: 0008-10-013 Supăort Piulita Axa Z.ipt:24 ↔ 0008-10-1004 Piulita.ipt:25
- Angle:25 (0 deg): 0008-10-008 X Axis suport.ipt:10 ↔ 0008-10-1013 LMK 10 Bearing.ipt:19
- Flush:121 (20 mm): 0008-10-1009 LM10uu.ipt:3 ↔ 0008-10-007 Contra suport injectomat.ipt:6
- Flush:122 (15 mm): 0008-10-007 Contra suport injectomat.ipt:6 ↔ 0008-10-1009 LM10uu.ipt:12
- Mate:188: 0008-10-1008 Bara 10_V1.ipt:8 ↔ 0008-10-010 Fixare AxaX.ipt:29
- Angle:28 (0 deg): 0008-10-009 X Axis suport.ipt:9 ↔ 0008-10-010 Fixare AxaX.ipt:29
- Flush:127: 0008-10-009 X Axis suport.ipt:9 ↔ 0008-10-010 Fixare AxaX.ipt:29
- Mate:189: 0008-10-1008 Bara 10_V1.ipt:8 ↔ 0008-10-010 Fixare AxaX.ipt:30
- Mate:190 (10 mm): 0008-10-010 Fixare AxaX.ipt:29 ↔ 0008-10-010 Fixare AxaX.ipt:30
- Mate:191: 0008-10-1008 Bara 10_V1.ipt:8 ↔ 0008-10-010 Fixare AxaX.ipt:31
- Angle:29 (0 deg): 0008-10-008 X Axis suport.ipt:10 ↔ 0008-10-010 Fixare AxaX.ipt:31
- Flush:128: 0008-10-008 X Axis suport.ipt:10 ↔ 0008-10-010 Fixare AxaX.ipt:31
- Mate:192: 0008-10-1008 Bara 10_V1.ipt:8 ↔ 0008-10-010 Fixare AxaX.ipt:32
- Flush:129: 0008-10-010 Fixare AxaX.ipt:31 ↔ 0008-10-010 Fixare AxaX.ipt:32
- Mate:193 (10 mm): 0008-10-010 Fixare AxaX.ipt:31 ↔ 0008-10-010 Fixare AxaX.ipt:32
- Angle:30 (0 deg): 0008-10-008 X Axis suport.ipt:10 ↔ 0008-10-012 Intinzator X.ipt:15
- Mate:194: 0008-10-009 X Axis suport.ipt:9 ↔ 0008-10-1013 LMK 10 Bearing.ipt:20
- Insert:22: 0008-10-2000 DIN 6912 - M4 x 25.ipt:120 ↔ 0008-10-2002 DIN 125 - A 4.3.ipt:121
- Insert:23: 0008-10-1013 LMK 10 Bearing.ipt:20 ↔ 0008-10-2002 DIN 125 - A 4.3.ipt:121
- Insert:24: 0008-10-2002 DIN 125 - A 4.3.ipt:122 ↔ 0008-10-2001 DIN 934 - M4 x 0.7.ipt:123
- Insert:25 (3.8 mm): 0008-10-2000 DIN 6912 - M4 x 25.ipt:120 ↔ 0008-10-2001 DIN 934 - M4 x 0.7.ipt:123
- [Insert]: 0008-10-2000 DIN 6912 - M4 x 25.ipt:124 ↔ 0008-10-2002 DIN 125 - A 4.3.ipt:125
- [Insert]: 0008-10-2002 DIN 125 - A 4.3.ipt:126 ↔ 0008-10-2001 DIN 934 - M4 x 0.7.ipt:127
- [Insert] (3.8 mm): 0008-10-2000 DIN 6912 - M4 x 25.ipt:124 ↔ 0008-10-2001 DIN 934 - M4 x 0.7.ipt:127
- Mate:195: 0008-10-1013 LMK 10 Bearing.ipt:20 ↔ 0008-10-2002 DIN 125 - A 4.3.ipt:125
- [Insert]: 0008-10-2000 DIN 6912 - M4 x 25.ipt:128 ↔ 0008-10-2002 DIN 125 - A 4.3.ipt:129
- [Insert]: 0008-10-2002 DIN 125 - A 4.3.ipt:130 ↔ 0008-10-2001 DIN 934 - M4 x 0.7.ipt:131
- [Insert] (3.8 mm): 0008-10-2000 DIN 6912 - M4 x 25.ipt:128 ↔ 0008-10-2001 DIN 934 - M4 x 0.7.ipt:131
- [Insert]: 0008-10-2000 DIN 6912 - M4 x 25.ipt:132 ↔ 0008-10-2002 DIN 125 - A 4.3.ipt:133
- [Insert]: 0008-10-2002 DIN 125 - A 4.3.ipt:134 ↔ 0008-10-2001 DIN 934 - M4 x 0.7.ipt:135
- [Insert] (3.8 mm): 0008-10-2000 DIN 6912 - M4 x 25.ipt:132 ↔ 0008-10-2001 DIN 934 - M4 x 0.7.ipt:135
- Insert:35: 0008-10-1013 LMK 10 Bearing.ipt:20 ↔ 0008-10-2002 DIN 125 - A 4.3.ipt:133
- Insert:36: 0008-10-1013 LMK 10 Bearing.ipt:20 ↔ 0008-10-2002 DIN 125 - A 4.3.ipt:129
- [Insert]: 0008-10-2000 DIN 6912 - M4 x 25.ipt:136 ↔ 0008-10-2002 DIN 125 - A 4.3.ipt:137
- [Insert]: 0008-10-2002 DIN 125 - A 4.3.ipt:138 ↔ 0008-10-2001 DIN 934 - M4 x 0.7.ipt:139
- [Insert] (3.8 mm): 0008-10-2000 DIN 6912 - M4 x 25.ipt:136 ↔ 0008-10-2001 DIN 934 - M4 x 0.7.ipt:139
- [Insert]: 0008-10-2000 DIN 6912 - M4 x 25.ipt:140 ↔ 0008-10-2002 DIN 125 - A 4.3.ipt:141
- [Insert]: 0008-10-2002 DIN 125 - A 4.3.ipt:142 ↔ 0008-10-2001 DIN 934 - M4 x 0.7.ipt:143
- [Insert] (3.8 mm): 0008-10-2000 DIN 6912 - M4 x 25.ipt:140 ↔ 0008-10-2001 DIN 934 - M4 x 0.7.ipt:143
- [Insert]: 0008-10-2000 DIN 6912 - M4 x 25.ipt:144 ↔ 0008-10-2002 DIN 125 - A 4.3.ipt:145
- [Insert]: 0008-10-2002 DIN 125 - A 4.3.ipt:146 ↔ 0008-10-2001 DIN 934 - M4 x 0.7.ipt:147
- [Insert] (3.8 mm): 0008-10-2000 DIN 6912 - M4 x 25.ipt:144 ↔ 0008-10-2001 DIN 934 - M4 x 0.7.ipt:147
- [Insert]: 0008-10-2000 DIN 6912 - M4 x 25.ipt:148 ↔ 0008-10-2002 DIN 125 - A 4.3.ipt:149
- [Insert]: 0008-10-2002 DIN 125 - A 4.3.ipt:150 ↔ 0008-10-2001 DIN 934 - M4 x 0.7.ipt:151
- [Insert] (3.8 mm): 0008-10-2000 DIN 6912 - M4 x 25.ipt:148 ↔ 0008-10-2001 DIN 934 - M4 x 0.7.ipt:151
- Insert:49: 0008-10-009 X Axis suport.ipt:9 ↔ 0008-10-2002 DIN 125 - A 4.3.ipt:149
- Insert:50: 0008-10-009 X Axis suport.ipt:9 ↔ 0008-10-2002 DIN 125 - A 4.3.ipt:137
- Insert:51: 0008-10-009 X Axis suport.ipt:9 ↔ 0008-10-2002 DIN 125 - A 4.3.ipt:145
- Insert:52: 0008-10-009 X Axis suport.ipt:9 ↔ 0008-10-2002 DIN 125 - A 4.3.ipt:141
- [Insert]: 0008-10-2000 DIN 6912 - M4 x 25.ipt:152 ↔ 0008-10-2002 DIN 125 - A 4.3.ipt:153
- [Insert]: 0008-10-2002 DIN 125 - A 4.3.ipt:154 ↔ 0008-10-2001 DIN 934 - M4 x 0.7.ipt:155
- [Insert] (3.8 mm): 0008-10-2000 DIN 6912 - M4 x 25.ipt:152 ↔ 0008-10-2001 DIN 934 - M4 x 0.7.ipt:155
- [Insert]: 0008-10-2000 DIN 6912 - M4 x 25.ipt:156 ↔ 0008-10-2002 DIN 125 - A 4.3.ipt:157
- [Insert]: 0008-10-2002 DIN 125 - A 4.3.ipt:158 ↔ 0008-10-2001 DIN 934 - M4 x 0.7.ipt:159
- [Insert] (3.8 mm): 0008-10-2000 DIN 6912 - M4 x 25.ipt:156 ↔ 0008-10-2001 DIN 934 - M4 x 0.7.ipt:159
- [Insert]: 0008-10-2000 DIN 6912 - M4 x 25.ipt:160 ↔ 0008-10-2002 DIN 125 - A 4.3.ipt:161
- [Insert]: 0008-10-2002 DIN 125 - A 4.3.ipt:162 ↔ 0008-10-2001 DIN 934 - M4 x 0.7.ipt:163
- [Insert] (3.8 mm): 0008-10-2000 DIN 6912 - M4 x 25.ipt:160 ↔ 0008-10-2001 DIN 934 - M4 x 0.7.ipt:163
- [Insert]: 0008-10-2000 DIN 6912 - M4 x 25.ipt:164 ↔ 0008-10-2002 DIN 125 - A 4.3.ipt:165
- [Insert]: 0008-10-2002 DIN 125 - A 4.3.ipt:166 ↔ 0008-10-2001 DIN 934 - M4 x 0.7.ipt:167
- [Insert] (3.8 mm): 0008-10-2000 DIN 6912 - M4 x 25.ipt:164 ↔ 0008-10-2001 DIN 934 - M4 x 0.7.ipt:167
- Insert:65: 0008-10-008 X Axis suport.ipt:10 ↔ 0008-10-2002 DIN 125 - A 4.3.ipt:157
- Insert:66: 0008-10-008 X Axis suport.ipt:10 ↔ 0008-10-2002 DIN 125 - A 4.3.ipt:153
- Insert:67: 0008-10-008 X Axis suport.ipt:10 ↔ 0008-10-2002 DIN 125 - A 4.3.ipt:161
- Insert:68: 0008-10-008 X Axis suport.ipt:10 ↔ 0008-10-2002 DIN 125 - A 4.3.ipt:165
- [Insert]: 0008-10-2000 DIN 6912 - M4 x 25.ipt:168 ↔ 0008-10-2002 DIN 125 - A 4.3.ipt:169
- [Insert]: 0008-10-2002 DIN 125 - A 4.3.ipt:170 ↔ 0008-10-2001 DIN 934 - M4 x 0.7.ipt:171
- [Insert] (3.8 mm): 0008-10-2000 DIN 6912 - M4 x 25.ipt:168 ↔ 0008-10-2001 DIN 934 - M4 x 0.7.ipt:171
- [Insert]: 0008-10-2000 DIN 6912 - M4 x 25.ipt:172 ↔ 0008-10-2002 DIN 125 - A 4.3.ipt:173
- [Insert]: 0008-10-2002 DIN 125 - A 4.3.ipt:174 ↔ 0008-10-2001 DIN 934 - M4 x 0.7.ipt:175
- [Insert] (3.8 mm): 0008-10-2000 DIN 6912 - M4 x 25.ipt:172 ↔ 0008-10-2001 DIN 934 - M4 x 0.7.ipt:175
- [Insert]: 0008-10-2000 DIN 6912 - M4 x 25.ipt:176 ↔ 0008-10-2002 DIN 125 - A 4.3.ipt:177
- [Insert]: 0008-10-2002 DIN 125 - A 4.3.ipt:178 ↔ 0008-10-2001 DIN 934 - M4 x 0.7.ipt:179
- [Insert] (3.8 mm): 0008-10-2000 DIN 6912 - M4 x 25.ipt:176 ↔ 0008-10-2001 DIN 934 - M4 x 0.7.ipt:179
- [Insert]: 0008-10-2000 DIN 6912 - M4 x 25.ipt:180 ↔ 0008-10-2002 DIN 125 - A 4.3.ipt:181
- [Insert]: 0008-10-2002 DIN 125 - A 4.3.ipt:182 ↔ 0008-10-2001 DIN 934 - M4 x 0.7.ipt:183
- [Insert] (3.8 mm): 0008-10-2000 DIN 6912 - M4 x 25.ipt:180 ↔ 0008-10-2001 DIN 934 - M4 x 0.7.ipt:183
- Insert:81: 0008-10-1013 LMK 10 Bearing.ipt:19 ↔ 0008-10-2002 DIN 125 - A 4.3.ipt:181
- Insert:82: 0008-10-1013 LMK 10 Bearing.ipt:19 ↔ 0008-10-2002 DIN 125 - A 4.3.ipt:177
- Insert:83: 0008-10-1013 LMK 10 Bearing.ipt:19 ↔ 0008-10-2002 DIN 125 - A 4.3.ipt:173
- Insert:84: 0008-10-1013 LMK 10 Bearing.ipt:19 ↔ 0008-10-2002 DIN 125 - A 4.3.ipt:169
- [Insert]: 0008-10-2002 DIN 125 - A 4.3.ipt:185 ↔ 0008-10-2001 DIN 934 - M4 x 0.7.ipt:186
- Insert:86: 0008-10-2018 DIN 912 - M4 x 0.7 x 40.ipt:184 ↔ 0008-10-2002 DIN 125 - A 4.3.ipt:187
- Insert:87 (2 mm): 0008-10-2018 DIN 912 - M4 x 0.7 x 40.ipt:184 ↔ 0008-10-2001 DIN 934 - M4 x 0.7.ipt:186
- Mate:196: 0008-10-008 X Axis suport.ipt:10 ↔ 0008-10-2002 DIN 125 - A 4.3.ipt:187
- [Insert]: 0008-10-2002 DIN 125 - A 4.3.ipt:189 ↔ 0008-10-2001 DIN 934 - M4 x 0.7.ipt:190
- [Insert]: 0008-10-2018 DIN 912 - M4 x 0.7 x 40.ipt:188 ↔ 0008-10-2002 DIN 125 - A 4.3.ipt:191
- [Insert] (2 mm): 0008-10-2018 DIN 912 - M4 x 0.7 x 40.ipt:188 ↔ 0008-10-2001 DIN 934 - M4 x 0.7.ipt:190
- Insert:91: 0008-10-008 X Axis suport.ipt:10 ↔ 0008-10-2002 DIN 125 - A 4.3.ipt:191
- [Insert]: 0008-10-2002 DIN 125 - A 4.3.ipt:193 ↔ 0008-10-2001 DIN 934 - M4 x 0.7.ipt:194
- [Insert]: 0008-10-2018 DIN 912 - M4 x 0.7 x 40.ipt:192 ↔ 0008-10-2002 DIN 125 - A 4.3.ipt:195
- [Insert] (2 mm): 0008-10-2018 DIN 912 - M4 x 0.7 x 40.ipt:192 ↔ 0008-10-2001 DIN 934 - M4 x 0.7.ipt:194
- [Insert]: 0008-10-2002 DIN 125 - A 4.3.ipt:197 ↔ 0008-10-2001 DIN 934 - M4 x 0.7.ipt:198
- [Insert]: 0008-10-2018 DIN 912 - M4 x 0.7 x 40.ipt:196 ↔ 0008-10-2002 DIN 125 - A 4.3.ipt:199
- [Insert] (2 mm): 0008-10-2018 DIN 912 - M4 x 0.7 x 40.ipt:196 ↔ 0008-10-2001 DIN 934 - M4 x 0.7.ipt:198
- Insert:98: 0008-10-008 X Axis suport.ipt:10 ↔ 0008-10-2002 DIN 125 - A 4.3.ipt:195
- Insert:99: 0008-10-008 X Axis suport.ipt:10 ↔ 0008-10-2002 DIN 125 - A 4.3.ipt:199
- [Insert]: 0008-10-2002 DIN 125 - A 4.3.ipt:201 ↔ 0008-10-2001 DIN 934 - M4 x 0.7.ipt:202
- [Insert]: 0008-10-2018 DIN 912 - M4 x 0.7 x 40.ipt:200 ↔ 0008-10-2002 DIN 125 - A 4.3.ipt:203
- [Insert] (2 mm): 0008-10-2018 DIN 912 - M4 x 0.7 x 40.ipt:200 ↔ 0008-10-2001 DIN 934 - M4 x 0.7.ipt:202
- [Insert]: 0008-10-2002 DIN 125 - A 4.3.ipt:205 ↔ 0008-10-2001 DIN 934 - M4 x 0.7.ipt:206
- [Insert]: 0008-10-2018 DIN 912 - M4 x 0.7 x 40.ipt:204 ↔ 0008-10-2002 DIN 125 - A 4.3.ipt:207
- [Insert] (2 mm): 0008-10-2018 DIN 912 - M4 x 0.7 x 40.ipt:204 ↔ 0008-10-2001 DIN 934 - M4 x 0.7.ipt:206
- [Insert]: 0008-10-2002 DIN 125 - A 4.3.ipt:209 ↔ 0008-10-2001 DIN 934 - M4 x 0.7.ipt:210
- [Insert]: 0008-10-2018 DIN 912 - M4 x 0.7 x 40.ipt:208 ↔ 0008-10-2002 DIN 125 - A 4.3.ipt:211
- [Insert] (2 mm): 0008-10-2018 DIN 912 - M4 x 0.7 x 40.ipt:208 ↔ 0008-10-2001 DIN 934 - M4 x 0.7.ipt:210
- Insert:109: 0008-10-008 X Axis suport.ipt:10 ↔ 0008-10-2002 DIN 125 - A 4.3.ipt:211
- Insert:110: 0008-10-008 X Axis suport.ipt:10 ↔ 0008-10-2002 DIN 125 - A 4.3.ipt:203
- Insert:111: 0008-10-008 X Axis suport.ipt:10 ↔ 0008-10-2002 DIN 125 - A 4.3.ipt:207
- [Insert]: 0008-10-2002 DIN 125 - A 4.3.ipt:213 ↔ 0008-10-2001 DIN 934 - M4 x 0.7.ipt:214
- [Insert]: 0008-10-2018 DIN 912 - M4 x 0.7 x 40.ipt:212 ↔ 0008-10-2002 DIN 125 - A 4.3.ipt:215
- [Insert] (2 mm): 0008-10-2018 DIN 912 - M4 x 0.7 x 40.ipt:212 ↔ 0008-10-2001 DIN 934 - M4 x 0.7.ipt:214
- [Insert]: 0008-10-2002 DIN 125 - A 4.3.ipt:217 ↔ 0008-10-2001 DIN 934 - M4 x 0.7.ipt:218
- [Insert]: 0008-10-2018 DIN 912 - M4 x 0.7 x 40.ipt:216 ↔ 0008-10-2002 DIN 125 - A 4.3.ipt:219
- [Insert] (2 mm): 0008-10-2018 DIN 912 - M4 x 0.7 x 40.ipt:216 ↔ 0008-10-2001 DIN 934 - M4 x 0.7.ipt:218
- [Insert]: 0008-10-2002 DIN 125 - A 4.3.ipt:221 ↔ 0008-10-2001 DIN 934 - M4 x 0.7.ipt:222
- [Insert]: 0008-10-2018 DIN 912 - M4 x 0.7 x 40.ipt:220 ↔ 0008-10-2002 DIN 125 - A 4.3.ipt:223